# Autodesk Inventor assembly: Asamblare
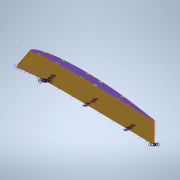
[picture p0: Inventor's stored thumbnail of the model, 180x180]
Saved by Autodesk Inventor 2022 (Build 260153000, 153)
## iProperties
Created: 2022-05-27
Part Number: Asamblare
Document SubType Name: Assembly
Designer: 40742
Title: Perfection
Author: 40742
## Documents named in this file (5)
- C:\Users\40742\Documents\Inventor\TASD\Asamblare.iam
- C:\Users\40742\Documents\Inventor\TASD\lonjeron.ipt
- C:\Users\40742\Documents\Inventor\TASD\Nervuri.ipt
- C:\Users\40742\Documents\Inventor\TASD\Lise (2).ipt
- C:\Users\40742\Documents\Inventor\TASD\Invelis.ipt
## Components (4 placed, 1 different names)
1. Profil:1 — Mate:1, Flush:1, Flush:2, Rigid:1
2. Profil:2 — Mate:1, Flush:1, Flush:2, Flush:3, Flush:4
3. Profil:3 — Flush:3
4. Profil:4 — Flush:4, Rigid:1
## Relationships (6: Flush 4, Mate 1, WeldJoint 1)
- Mate:1: Profil:1 ↔ Profil:2
- Flush:1: Profil:1 ↔ Profil:2
- Flush:2: Profil:1 ↔ Profil:2
- Flush:3: Profil:2 ↔ Profil:3
- Flush:4: Profil:2 ↔ Profil:4
- Rigid:1 [WeldJoint]: Profil:1 ↔ Profil:4
